# Autodesk Inventor assembly: gauge_with_cleat
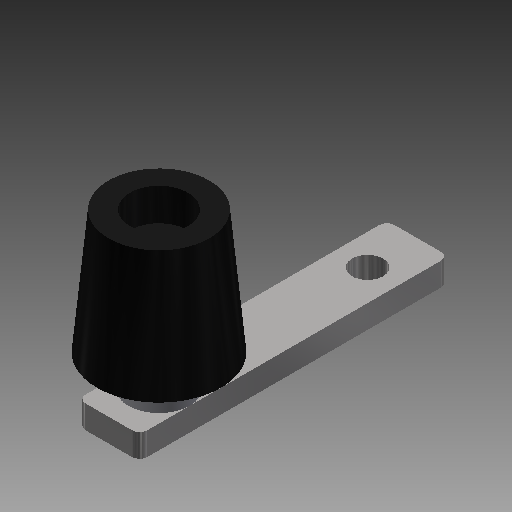
[picture p0: Inventor's stored thumbnail of the model, 512x512]
Saved by Autodesk Inventor 2018 (Build 220112000, 112)
## iProperties
Created: 2018-05-01
Part Number: gauge_with_cleat
Document SubType Name: Assembly
Designer: medrimonia
Author: medrimonia
## Documents named in this file (4)
- C:\Users\etd\Dropbox\SigmaBan\SigmaBanV2.1\gauge_with_cleat.iam
- C:\Users\etd\Dropbox\SigmaBan\SigmaBanV2.1\gauge.ipt
- C:\Users\etd\Dropbox\SigmaBan\SigmaBanV2.1\gauge_ring.ipt
- C:\Users\etd\Dropbox\SigmaBan\SigmaBanV2.1\cleat.ipt
## Components (3 placed, 3 different names)
1. gauge:1 — Mate:1, Mate:2
2. gauge_ring:1 — Mate:1, Mate:2, Mate:3, Mate:4
3. cleat:1 — Mate:3, Mate:4
## Relationships (4: Mate 4)
- Mate:1: gauge:1 ↔ gauge_ring:1
- Mate:2: gauge:1 ↔ gauge_ring:1
- Mate:3: gauge_ring:1 ↔ cleat:1
- Mate:4: gauge_ring:1 ↔ cleat:1
